# Autodesk Inventor assembly: Outer
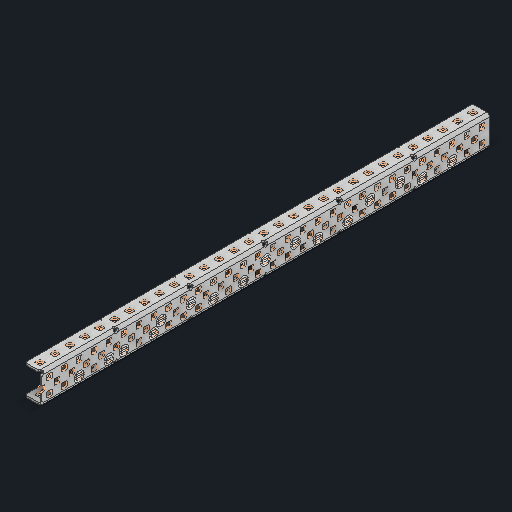
[picture p0: Inventor's stored thumbnail of the model, 512x512]
Saved by Autodesk Inventor 2025.1 (Build 291241000, 241)
## iProperties
Created: 2024-11-01
Part Number: Outer
Document SubType Name: Assembly
Designer: avere
Author: avere
## Documents named in this file (3)
- C:\Users\avere\VEX\High Stakes\CAD\V2\Chassis V2\Drivebay Left\Outer.iam
- C:\Users\avere\VEX\High Stakes\CAD\ROBOPROS-CAD-Inventor\Structure\C Channel\Aluminum 1x2x1\Alu C 1x2x1x30.ipt
- C:\Users\avere\VEX\High Stakes\CAD\ROBOPROS-CAD-Inventor\Quick Assemblies\Bearing Flat NScrew Slotted.iam
## Components (9 placed, 2 different names)
1. Alu C 1x2x1x30:1 — Mate:1, Flush:3, Flush:4, Insert:5, Mate:6, Insert:6, Mate:7, Insert:7, Mate:8, Insert:8, Mate:9
2. Bearing Flat NScrew Slotted:7 [sub-assembly] — Insert:5, Mate:6
3. Bearing Flat NScrew Slotted:8 [sub-assembly] — Insert:6, Mate:7
4. Bearing Flat NScrew Slotted:9 [sub-assembly] — Insert:8, Mate:9
5. Bearing Flat NScrew Slotted:10 [sub-assembly]
6. Bearing Flat NScrew Slotted:11 [sub-assembly]
7. Bearing Flat NScrew Slotted:3 [sub-assembly] — Insert:7, Mate:8
8. Bearing Flat NScrew Slotted:12 [sub-assembly]
9. Bearing Flat NScrew Slotted:13 [sub-assembly]
## Component patterns: (3 elements, first: Bearing Flat NScrew Slotted:9), (3 elements, first: Bearing Flat NScrew Slotted:3)
## Relationships (11: Mate 5, Insert 4, Flush 2)
- Mate:1 (-190.5 mm): Alu C 1x2x1x30:1
- Flush:3 (-12.7 mm): Alu C 1x2x1x30:1
- Flush:4 (-7.9375 mm): Alu C 1x2x1x30:1
- Insert:5: Alu C 1x2x1x30:1 ↔ Bearing Flat NScrew Slotted:7
- Mate:6: Alu C 1x2x1x30:1 ↔ Bearing Flat NScrew Slotted:7
- Insert:6: Alu C 1x2x1x30:1 ↔ Bearing Flat NScrew Slotted:8
- Mate:7: Alu C 1x2x1x30:1 ↔ Bearing Flat NScrew Slotted:8
- Insert:7: Alu C 1x2x1x30:1 ↔ Bearing Flat NScrew Slotted:3
- Mate:8: Alu C 1x2x1x30:1 ↔ Bearing Flat NScrew Slotted:3
- Insert:8: Alu C 1x2x1x30:1 ↔ Bearing Flat NScrew Slotted:9
- Mate:9: Alu C 1x2x1x30:1 ↔ Bearing Flat NScrew Slotted:9
